# Autodesk Inventor assembly: pulley .25 in + wheel.2
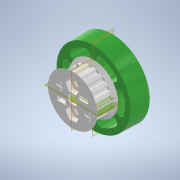
[picture p0: Inventor's stored thumbnail of the model, 180x180]
Saved by Autodesk Inventor 2020 (Build 240168000, 168)
## iProperties
Created: 2020-01-23
Part Number: pulley .25 in + wheel.2
Document SubType Name: Assembly
Designer: jackm
Author: jackm
## Documents named in this file (3)
- D:\FTC8863\2019 Robot\general robot componets\pulley .25 in + wheel.2.iam
- D:\FTC8863\Andymark\am-3572 2IN 8mm Compliant Wheel REV2.ipt
- D:\FTC8863\2019 Robot\Generic Parts\18 tooth .2 pitch pulley .25 in D bore assembled from halves.iam
## Components (2 placed, 2 different names)
1. am-3572 2IN 8mm Compliant Wheel REV2:1 — Mate:1, Mate:2
2. 18 tooth .2 pitch pulley .25 in D bore assembled from halves:1 [sub-assembly] — Mate:1, Mate:2
## Relationships (2: Mate 2)
- Mate:1: am-3572 2IN 8mm Compliant Wheel REV2:1 ↔ 18 tooth .2 pitch pulley .25 in D bore assembled from halves:1
- Mate:2: am-3572 2IN 8mm Compliant Wheel REV2:1 ↔ 18 tooth .2 pitch pulley .25 in D bore assembled from halves:1
